# Autodesk Inventor assembly: ENCORDER_UNIT_LEFT_sa
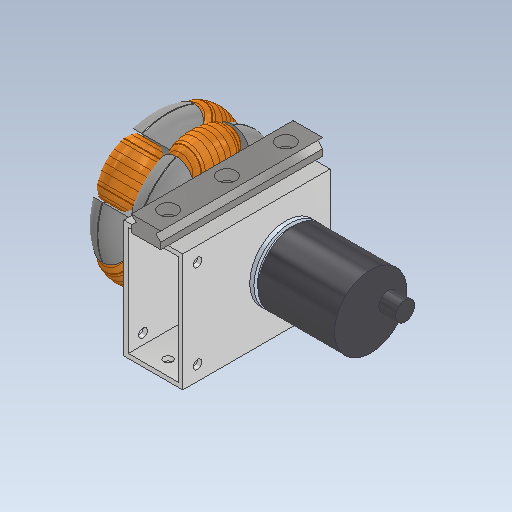
[picture p0: Inventor's stored thumbnail of the model, 512x512]
Saved by Autodesk Inventor 2020 (Build 240168000, 168)
## iProperties
Created: 2019-06-15
Part Number: ENCORDER_UNIT_LEFT_sa
Document SubType Name: Assembly
Designer: shun
Author: shun
## Documents named in this file (8)
- C:\Users\shun\Documents\Inventor\3wheel_omuni_2019\接地エンコーダーユニット\あ\ENCORDER_UNIT_LEFT_sa.iam
- C:\Users\shun\Documents\Inventor\3wheel_omuni_2019\接地エンコーダーユニット\あ\LINEAR_GUIDE_SSEB10_55_KH.ipt
- C:\Users\shun\Documents\Inventor\3wheel_omuni_2019\接地エンコーダーユニット\あ\K20X40X1P5_50_ENC_KH.ipt
- C:\Users\shun\Documents\Inventor\3wheel_omuni_2019\接地エンコーダーユニット\あ\ENCORDER_KH.ipt
- C:\Users\shun\Documents\Inventor\3wheel_omuni_2019\接地エンコーダーユニット\あ\BEAR_F13P8_12_8_ENC_KH.ipt
- C:\Users\shun\Documents\Inventor\3wheel_omuni_2019\接地エンコーダーユニット\あ\SPACER_14_8_2_ENC_KH.ipt
- C:\Users\shun\Documents\Inventor\3wheel_omuni_2019\接地エンコーダーユニット\あ\ROTACASTER_48_KH.iam
- C:\Users\shun\Documents\Inventor\3wheel_omuni_2019\接地エンコーダーユニット\あ\S14P9_45_ENC_KH.ipt
## Components (7 placed, 7 different names)
1. LINEAR_GUIDE_SSEB10_55_KH:1 — 挿入:1, メイト:1
2. K20X40X1P5_50_ENC_KH:1 — 挿入:1, メイト:1, 挿入:2, メイト:2, 挿入:3
3. ENCORDER_KH:1 — 挿入:2, メイト:2
4. BEAR_F13P8_12_8_ENC_KH:1 — 挿入:3, 挿入:4
5. SPACER_14_8_2_ENC_KH:1 — 挿入:4, 挿入:5
6. ROTACASTER_48_KH:1 [sub-assembly] — 挿入:5, 挿入:6
7. S14P9_45_ENC_KH:1 — 挿入:6
## Relationships (8: Insert 6, Mate 2)
- 挿入:1 [Insert]: LINEAR_GUIDE_SSEB10_55_KH:1 ↔ K20X40X1P5_50_ENC_KH:1
- メイト:1 [Mate]: LINEAR_GUIDE_SSEB10_55_KH:1 ↔ K20X40X1P5_50_ENC_KH:1
- 挿入:2 [Insert]: K20X40X1P5_50_ENC_KH:1 ↔ ENCORDER_KH:1
- メイト:2 [Mate]: K20X40X1P5_50_ENC_KH:1 ↔ ENCORDER_KH:1
- 挿入:3 [Insert]: K20X40X1P5_50_ENC_KH:1 ↔ BEAR_F13P8_12_8_ENC_KH:1
- 挿入:4 [Insert]: BEAR_F13P8_12_8_ENC_KH:1 ↔ SPACER_14_8_2_ENC_KH:1
- 挿入:5 [Insert]: SPACER_14_8_2_ENC_KH:1 ↔ ROTACASTER_48_KH:1
- 挿入:6 [Insert]: ROTACASTER_48_KH:1 ↔ S14P9_45_ENC_KH:1
